# Autodesk Inventor assembly: Assembly2
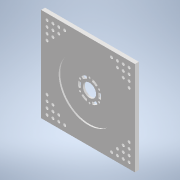
[picture p0: Inventor's stored thumbnail of the model, 180x180]
Saved by Autodesk Inventor 2020 (Build 240168000, 168)
## iProperties
Created: 2020-01-23
Part Number: Assembly2
Document SubType Name: Assembly
Designer: srini
Author: srini
## Documents named in this file (3)
- C:\Users\srini\Documents\FRC\2020\Assembly2.iam
- C:\Users\srini\Documents\FRC\2020\Tooling\60t_Aluminum_Plate_Sprocket_35_Chain_1-1_8_Bearing_Bore_217-2644.ipt
- C:\Users\srini\Documents\FRC\2020\IntakeShooter\60T-LocatorPlate.ipt
## Components (2 placed, 2 different names)
1. 60t_Aluminum_Plate_Sprocket_35_Chain_1-1_8_Bearing_Bore_217-2644:1 — Flush:1
2. 60T-LocatorPlate:1 — Flush:1
## Relationships (1: Flush 1)
- Flush:1: 60t_Aluminum_Plate_Sprocket_35_Chain_1-1_8_Bearing_Bore_217-2644:1 ↔ 60T-LocatorPlate:1
